# Autodesk Inventor assembly: enc-SidePanel Links Unten
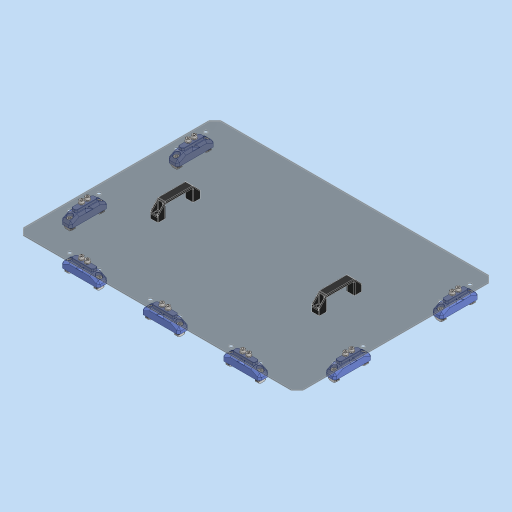
[picture p0: Inventor's stored thumbnail of the model, 512x512]
Saved by Autodesk Inventor 2023.2 (Build 272271000, 271)
## iProperties
Created: 2023-11-30
Part Number: enc-SidePanel Links Unten
Document SubType Name: Assembly
Designer: Nils Bade
Author: Nils Bade
## Documents named in this file (5)
- C:\Users\nilsb\Documents\Inventor\Projektarbeit-Bade\Enclosure\enc-SidePanel Links Unten.iam
- C:\Users\nilsb\Documents\Inventor\Projektarbeit-Bade\Enclosure\enc-SidePanel 500x708.ipt
- C:\Users\nilsb\Documents\Inventor\Projektarbeit-Bade\Enclosure\V-Slot Door Handle v1.ipt
- C:\Users\nilsb\Documents\Inventor\Projektarbeit-Bade\Enclosure\Magnet Panel for 4040 - Assembly.iam
- C:\Users\nilsb\Documents\Inventor\Projektarbeit-Bade\Enclosure\Magnet Frame Straight for 4040 - Assembly.iam
## Components (17 placed, 4 different names)
1. enc-SidePanel Unten 500x708:1 — Passend:1, Passend:2, Passend:3, Passend:4, Passend:5, Passend:6, Passend:7, Passend:8, Passend:9, Passend:10, Passend:11, Passend:12, Passend:13, Passend:14, Passend:15, Passend:16, Passend:17, Passend:18, Passend:19, Passend:20, Passend:21, Passend:22, Passend:23, Passend:24, Passend:25, Passend:39
2. V-Slot Door Handle v1:1 — Passend:1, Passend:2, Passend:6
3. V-Slot Door Handle v1:2 — Passend:3, Passend:4, Passend:5
4. Magnet Panel for 4040 - Assembly:1 [sub-assembly] — Passend:7, Passend:8, Passend:9, Passend:35, Passend:44, Passend:45
5. Magnet Panel for 4040 - Assembly:2 [sub-assembly] — Passend:10, Passend:11, Passend:12, Passend:36, Passend:46, Passend:47
6. Magnet Panel for 4040 - Assembly:3 [sub-assembly] — Passend:22, Passend:38, Passend:39, Passend:40, Passend:41
7. Magnet Panel for 4040 - Assembly:4 [sub-assembly] — Passend:23, Passend:24, Passend:25, Passend:37, Passend:42, Passend:43
8. Magnet Panel for 4040 - Assembly:5 [sub-assembly] — Passend:19, Passend:20, Passend:21, Passend:26, Passend:27, Passend:28
9. Magnet Panel for 4040 - Assembly:6 [sub-assembly] — Passend:16, Passend:17, Passend:18, Passend:29, Passend:31, Passend:34
10. Magnet Panel for 4040 - Assembly:7 [sub-assembly] — Passend:13, Passend:14, Passend:15, Passend:30, Passend:32, Passend:33
11. Magnet Frame Straight for 4040 - Assembly:1 [sub-assembly] — Passend:35, Passend:44, Passend:45
12. Magnet Frame Straight for 4040 - Assembly:2 [sub-assembly] — Passend:36, Passend:46, Passend:47
13. Magnet Frame Straight for 4040 - Assembly:3 [sub-assembly] — Passend:37, Passend:42, Passend:43
14. Magnet Frame Straight for 4040 - Assembly:4 [sub-assembly] — Passend:38, Passend:40, Passend:41
15. Magnet Frame Straight for 4040 - Assembly:5 [sub-assembly] — Passend:26, Passend:27, Passend:28
16. Magnet Frame Straight for 4040 - Assembly:6 [sub-assembly] — Passend:29, Passend:31, Passend:34
17. Magnet Frame Straight for 4040 - Assembly:7 [sub-assembly] — Passend:30, Passend:32, Passend:33
## Relationships (47: Mate 47)
- Passend:1 [Mate]: enc-SidePanel Unten 500x708:1 ↔ V-Slot Door Handle v1:1
- Passend:2 [Mate]: enc-SidePanel Unten 500x708:1 ↔ V-Slot Door Handle v1:1
- Passend:3 [Mate]: enc-SidePanel Unten 500x708:1 ↔ V-Slot Door Handle v1:2
- Passend:4 [Mate]: enc-SidePanel Unten 500x708:1 ↔ V-Slot Door Handle v1:2
- Passend:5 [Mate]: enc-SidePanel Unten 500x708:1 ↔ V-Slot Door Handle v1:2
- Passend:6 [Mate]: enc-SidePanel Unten 500x708:1 ↔ V-Slot Door Handle v1:1
- Passend:7 [Mate]: enc-SidePanel Unten 500x708:1 ↔ Magnet Panel for 4040 - Assembly:1
- Passend:8 [Mate]: enc-SidePanel Unten 500x708:1 ↔ Magnet Panel for 4040 - Assembly:1
- Passend:9 [Mate]: enc-SidePanel Unten 500x708:1 ↔ Magnet Panel for 4040 - Assembly:1
- Passend:10 [Mate]: enc-SidePanel Unten 500x708:1 ↔ Magnet Panel for 4040 - Assembly:2
- Passend:11 [Mate]: enc-SidePanel Unten 500x708:1 ↔ Magnet Panel for 4040 - Assembly:2
- Passend:12 [Mate]: enc-SidePanel Unten 500x708:1 ↔ Magnet Panel for 4040 - Assembly:2
- Passend:13 [Mate]: enc-SidePanel Unten 500x708:1 ↔ Magnet Panel for 4040 - Assembly:7
- Passend:14 [Mate]: enc-SidePanel Unten 500x708:1 ↔ Magnet Panel for 4040 - Assembly:7
- Passend:15 [Mate]: enc-SidePanel Unten 500x708:1 ↔ Magnet Panel for 4040 - Assembly:7
- Passend:16 [Mate]: enc-SidePanel Unten 500x708:1 ↔ Magnet Panel for 4040 - Assembly:6
- Passend:17 [Mate]: enc-SidePanel Unten 500x708:1 ↔ Magnet Panel for 4040 - Assembly:6
- Passend:18 [Mate]: enc-SidePanel Unten 500x708:1 ↔ Magnet Panel for 4040 - Assembly:6
- Passend:19 [Mate]: enc-SidePanel Unten 500x708:1 ↔ Magnet Panel for 4040 - Assembly:5
- Passend:20 [Mate]: enc-SidePanel Unten 500x708:1 ↔ Magnet Panel for 4040 - Assembly:5
- Passend:21 [Mate]: enc-SidePanel Unten 500x708:1 ↔ Magnet Panel for 4040 - Assembly:5
- Passend:22 [Mate]: enc-SidePanel Unten 500x708:1 ↔ Magnet Panel for 4040 - Assembly:3
- Passend:23 [Mate]: enc-SidePanel Unten 500x708:1 ↔ Magnet Panel for 4040 - Assembly:4
- Passend:24 [Mate]: enc-SidePanel Unten 500x708:1 ↔ Magnet Panel for 4040 - Assembly:4
- Passend:25 [Mate]: enc-SidePanel Unten 500x708:1 ↔ Magnet Panel for 4040 - Assembly:4
- Passend:26 [Mate]: Magnet Panel for 4040 - Assembly:5 ↔ Magnet Frame Straight for 4040 - Assembly:5
- Passend:27 [Mate]: Magnet Panel for 4040 - Assembly:5 ↔ Magnet Frame Straight for 4040 - Assembly:5
- Passend:28 [Mate]: Magnet Panel for 4040 - Assembly:5 ↔ Magnet Frame Straight for 4040 - Assembly:5
- Passend:29 [Mate]: Magnet Panel for 4040 - Assembly:6 ↔ Magnet Frame Straight for 4040 - Assembly:6
- Passend:30 [Mate]: Magnet Panel for 4040 - Assembly:7 ↔ Magnet Frame Straight for 4040 - Assembly:7
- Passend:31 [Mate]: Magnet Panel for 4040 - Assembly:6 ↔ Magnet Frame Straight for 4040 - Assembly:6
- Passend:32 [Mate]: Magnet Panel for 4040 - Assembly:7 ↔ Magnet Frame Straight for 4040 - Assembly:7
- Passend:33 [Mate]: Magnet Panel for 4040 - Assembly:7 ↔ Magnet Frame Straight for 4040 - Assembly:7
- Passend:34 [Mate]: Magnet Panel for 4040 - Assembly:6 ↔ Magnet Frame Straight for 4040 - Assembly:6
- Passend:35 [Mate]: Magnet Panel for 4040 - Assembly:1 ↔ Magnet Frame Straight for 4040 - Assembly:1
- Passend:36 [Mate]: Magnet Panel for 4040 - Assembly:2 ↔ Magnet Frame Straight for 4040 - Assembly:2
- Passend:37 [Mate]: Magnet Panel for 4040 - Assembly:4 ↔ Magnet Frame Straight for 4040 - Assembly:3
- Passend:38 [Mate]: Magnet Panel for 4040 - Assembly:3 ↔ Magnet Frame Straight for 4040 - Assembly:4
- Passend:39 [Mate]: enc-SidePanel Unten 500x708:1 ↔ Magnet Panel for 4040 - Assembly:3
- Passend:40 [Mate]: Magnet Panel for 4040 - Assembly:3 ↔ Magnet Frame Straight for 4040 - Assembly:4
- Passend:41 [Mate]: Magnet Panel for 4040 - Assembly:3 ↔ Magnet Frame Straight for 4040 - Assembly:4
- Passend:42 [Mate]: Magnet Panel for 4040 - Assembly:4 ↔ Magnet Frame Straight for 4040 - Assembly:3
- Passend:43 [Mate]: Magnet Panel for 4040 - Assembly:4 ↔ Magnet Frame Straight for 4040 - Assembly:3
- Passend:44 [Mate]: Magnet Panel for 4040 - Assembly:1 ↔ Magnet Frame Straight for 4040 - Assembly:1
- Passend:45 [Mate]: Magnet Panel for 4040 - Assembly:1 ↔ Magnet Frame Straight for 4040 - Assembly:1
- Passend:46 [Mate]: Magnet Panel for 4040 - Assembly:2 ↔ Magnet Frame Straight for 4040 - Assembly:2
- Passend:47 [Mate]: Magnet Panel for 4040 - Assembly:2 ↔ Magnet Frame Straight for 4040 - Assembly:2
